# Autodesk Inventor assembly: robot
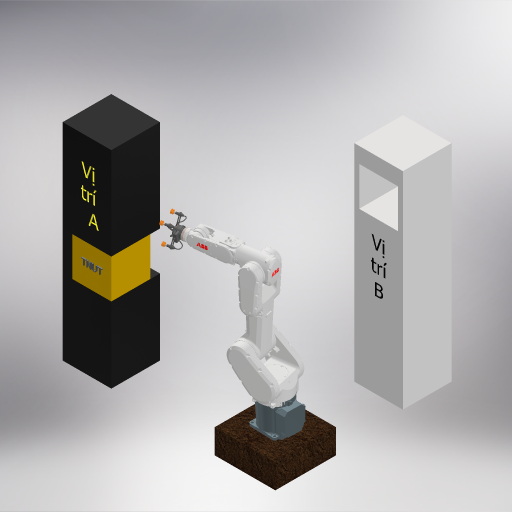
[picture p0: Inventor's stored thumbnail of the model, 512x512]
Saved by Autodesk Inventor 2023.3 (Build 273359000, 359)
## iProperties
Created: 2023-05-23
Part Number: robot
Document SubType Name: Assembly
Designer: Nguyen Xuan Lam
Author: Nguyen Xuan Lam
## Documents named in this file (11)
- C:\Users\Admin\Downloads\IRB 1300-1150_OmniCore_rev02_SAT_j\IRB 1300-1150_OmniCore_rev02_SAT_j\robot.iam
- C:\Users\Admin\Downloads\IRB 1300-1150_OmniCore_rev02_SAT_j\IRB 1300-1150_OmniCore_rev02_SAT_j\link0-bottom cable\link0-bottom cable.ipt
- C:\Users\Admin\Downloads\IRB 1300-1150_OmniCore_rev02_SAT_j\IRB 1300-1150_OmniCore_rev02_SAT_j\link1_1400\link1_1400.ipt
- C:\Users\Admin\Downloads\IRB 1300-1150_OmniCore_rev02_SAT_j\IRB 1300-1150_OmniCore_rev02_SAT_j\link2_1150\link2_1150.ipt
- C:\Users\Admin\Downloads\IRB 1300-1150_OmniCore_rev02_SAT_j\IRB 1300-1150_OmniCore_rev02_SAT_j\space.ipt
- C:\Users\Admin\Downloads\IRB 1300-1150_OmniCore_rev02_SAT_j\IRB 1300-1150_OmniCore_rev02_SAT_j\link4_900\link4_900.ipt
- C:\Users\Admin\Downloads\IRB 1300-1150_OmniCore_rev02_SAT_j\IRB 1300-1150_OmniCore_rev02_SAT_j\link3\link3.ipt
- C:\Users\Admin\Downloads\IRB 1300-1150_OmniCore_rev02_SAT_j\IRB 1300-1150_OmniCore_rev02_SAT_j\link5-foundry\link5-foundry.ipt
- C:\Users\Admin\Downloads\IRB 1300-1150_OmniCore_rev02_SAT_j\IRB 1300-1150_OmniCore_rev02_SAT_j\link6-foundry\link6-foundry.ipt
- C:\Users\Admin\Downloads\IRB 1300-1150_OmniCore_rev02_SAT_j\IRB 1300-1150_OmniCore_rev02_SAT_j\Part36.ipt
- C:\Users\Admin\Downloads\Vacuum gripper\Vacuum gripper.ipt
## Components (10 placed, 10 different names)
1. space:1 — Mate:3, Mate:4, Mate:21, Mate:22, Mate:23
2. link0-bottom cable:1 — Mate:1, Mate:2, Mate:3, Mate:4, q1
3. link1_1400:1 — Mate:1, Mate:2, Mate:6, Mate:17, q2, q1
4. link2_1150:1 — Mate:6, Mate:7, Mate:9, Mate:17, q2, q3
5. link3:1 — Mate:7, Mate:9, Mate:10, Mate:11, q3, q4
6. link4_900:1 — Mate:10, Mate:11, Mate:13, q4, Mate:24, q5
7. link5-foundry:1 — Mate:13, Mate:14, Mate:15, Angle:5, q5, q6, Mate:24
8. link6-foundry:3 — Mate:14, Mate:15, Mate:18, Mate:19
9. Part36:1 — Mate:20, Mate:21, Mate:22, Mate:23
10. Vacuum gripper:1 — Mate:18, Mate:19, Angle:5, q6, Mate:20
## Relationships (27: Mate 20, Angle 7)
- Mate:1 (-31.81 mm): link0-bottom cable:1 ↔ link1_1400:1
- Mate:2 (2.317 mm): link0-bottom cable:1 ↔ link1_1400:1
- Mate:3: space:1 ↔ link0-bottom cable:1
- Mate:6: link1_1400:1 ↔ link2_1150:1
- Mate:7: link2_1150:1 ↔ link3:1
- Mate:9: link2_1150:1 ↔ link3:1
- Mate:10: link3:1 ↔ link4_900:1
- Mate:11: link3:1 ↔ link4_900:1
- Mate:13: link4_900:1 ↔ link5-foundry:1
- Mate:14: link5-foundry:1 ↔ link6-foundry:3
- Mate:15: link5-foundry:1 ↔ link6-foundry:3
- Mate:17: link1_1400:1 ↔ link2_1150:1
- Mate:18: link6-foundry:3 ↔ Vacuum gripper:1
- Mate:19: link6-foundry:3 ↔ Vacuum gripper:1
- Angle:5 (180 deg): link5-foundry:1 ↔ Vacuum gripper:1
- Mate:4: space:1 ↔ link0-bottom cable:1
- q2 [Angle] (90 deg): link1_1400:1 ↔ link2_1150:1
- q3 [Angle] (90 deg): link2_1150:1 ↔ link3:1
- q5 [Angle] (3.25 deg): link4_900:1 ↔ link5-foundry:1
- q6 [Angle] (370 deg): link5-foundry:1 ↔ Vacuum gripper:1
- Mate:20 (128 mm): Part36:1 ↔ Vacuum gripper:1
- Mate:21: space:1 ↔ Part36:1
- Mate:22: space:1 ↔ Part36:1
- Mate:23: space:1 ↔ Part36:1
- q4 [Angle] (4.16 deg): link3:1 ↔ link4_900:1
- q1 [Angle] (4 deg): link0-bottom cable:1 ↔ link1_1400:1
- Mate:24: link4_900:1 ↔ link5-foundry:1
